# Autodesk Inventor assembly: Servo ModelMicroServo9g
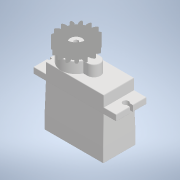
[picture p0: Inventor's stored thumbnail of the model, 180x180]
Saved by Autodesk Inventor 2020.2 (Build 242310000, 310)
## iProperties
Company: unknown
Created: 2013-08-04
Part Number: Servo ModelMicroServo9g
Document SubType Name: Assembly
Designer: othscs164
Sending System: unknown
Preprocessor: unknown
Minimum Resolution: 0.001
Sending System Product ID: MicroServo9g
Sent Units: Centimeter
Translation Standard: IGES 5.3
Title: MicroServo9g
Author: unknown
## Documents named in this file (3)
- C:\Users\Varun Kumar\Desktop\ServoArm\Servo ModelMicroServo9g.iam
- C:\Users\Varun Kumar\Desktop\ServoArm\Servo ModelPart16.ipt
- C:\Users\Varun Kumar\Desktop\ServoArm\CE3_Round_gear.ipt
## Components (2 placed, 2 different names)
1. Servo ModelPart16 — Mate:1, Mate:2
2. CE3_Round_gear:1 — Mate:1, Mate:2
## Relationships (2: Mate 2)
- Mate:1: Servo ModelPart16 ↔ CE3_Round_gear:1
- Mate:2: Servo ModelPart16 ↔ CE3_Round_gear:1
